# Autodesk Inventor assembly: Camera Box Assembly
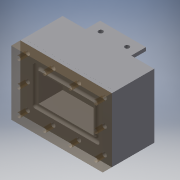
[picture p0: Inventor's stored thumbnail of the model, 180x180]
Saved by Autodesk Inventor 2018 (Build 220112000, 112)
## iProperties
Created: 2018-04-18
Part Number: Camera Box Assembly
Document SubType Name: Assembly
Designer: trent
Author: trent
## Documents named in this file (7)
- F:\RoboSub 2018\Camera\Camera Box Assembly.iam
- F:\RoboSub 2018\Camera\Front.ipt
- F:\RoboSub 2018\Camera\Side.ipt
- F:\RoboSub 2018\Camera\Top.ipt
- F:\RoboSub 2018\Camera\Bottom.ipt
- F:\RoboSub 2018\Camera\Back.ipt
- F:\RoboSub 2018\Camera\Acrylic Front.ipt
## Components (7 placed, 6 different names)
1. Front:1 — Mate:1, Flush:1, Mate:2, Mate:4, Mate:6, Flush:5, Mate:10
2. Side:2 — Mate:3, Mate:4, Flush:2, Mate:5, Flush:3, Flush:7
3. Top:1 — Mate:5, Flush:3, Mate:6, Mate:9, Flush:8
4. Bottom:1 — Mate:1, Flush:1, Mate:2, Mate:3, Flush:2, Mate:7, Flush:4, Flush:6
5. Side:3 — Mate:7, Flush:4, Flush:5, Mate:8
6. Back:1 — Mate:8, Flush:6, Mate:9
7. Acrylic Front:1 — Flush:7, Flush:8, Mate:10
## Relationships (18: Mate 10, Flush 8)
- Mate:1: Front:1 ↔ Bottom:1
- Flush:1: Front:1 ↔ Bottom:1
- Mate:2: Front:1 ↔ Bottom:1
- Mate:3: Side:2 ↔ Bottom:1
- Mate:4: Front:1 ↔ Side:2
- Flush:2: Side:2 ↔ Bottom:1
- Mate:5: Side:2 ↔ Top:1
- Flush:3: Side:2 ↔ Top:1
- Mate:6: Front:1 ↔ Top:1
- Mate:7: Bottom:1 ↔ Side:3
- Flush:4: Bottom:1 ↔ Side:3
- Flush:5: Front:1 ↔ Side:3
- Mate:8: Side:3 ↔ Back:1
- Flush:6: Bottom:1 ↔ Back:1
- Mate:9: Top:1 ↔ Back:1
- Flush:7: Side:2 ↔ Acrylic Front:1
- Flush:8: Top:1 ↔ Acrylic Front:1
- Mate:10: Front:1 ↔ Acrylic Front:1
